# Autodesk Inventor assembly: Assembly1
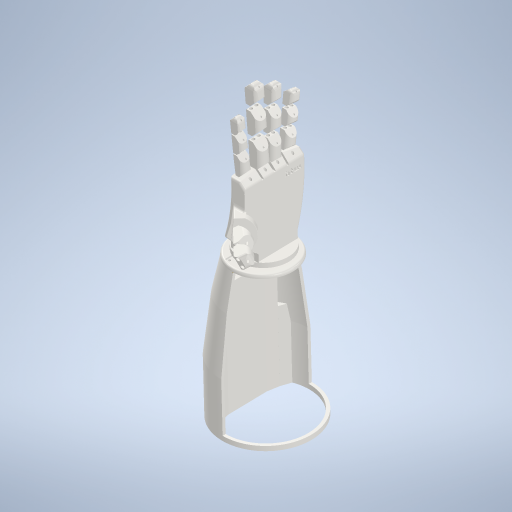
[picture p0: Inventor's stored thumbnail of the model, 512x512]
Saved by Autodesk Inventor 2024 (Build 280153000, 153)
## iProperties
Created: 2025-06-11
Part Number: Assembly1
Document SubType Name: Assembly
Designer: Mehdi Charfeddine
Author: Mehdi Charfeddine
## Documents named in this file (8)
- C:\Users\Mehdi Charfeddine\OneDrive\Bureau\original 3d\Assembly1.iam
- C:\Users\Mehdi Charfeddine\OneDrive\Bureau\original 3d\hand update.ipt
- C:\Users\Mehdi Charfeddine\OneDrive\Bureau\original 3d\update arm.ipt
- C:\Users\Mehdi Charfeddine\OneDrive\Bureau\original 3d\Daumen.ipt
- C:\Users\Mehdi Charfeddine\OneDrive\Bureau\original 3d\Zeigefinger.ipt
- C:\Users\Mehdi Charfeddine\OneDrive\Bureau\original 3d\Mittelfinger.ipt
- C:\Users\Mehdi Charfeddine\OneDrive\Bureau\original 3d\Ringfinger.ipt
- C:\Users\Mehdi Charfeddine\OneDrive\Bureau\original 3d\Kleiner Finger.ipt
## Components (7 placed, 7 different names)
1. hand update:1 — Mate:1, Mate:2, Mate:3, Mate:4, Mate:5, Mate:6
2. update arm:1 — Mate:1
3. Daumen:1 — Mate:2
4. Zeigefinger:1 — Mate:3
5. Mittelfinger:1 — Mate:4
6. Ringfinger:1 — Mate:5
7. Kleiner Finger:1 — Mate:6
## Relationships (6: Mate 6)
- Mate:1: hand update:1 ↔ update arm:1
- Mate:2: hand update:1 ↔ Daumen:1
- Mate:3: hand update:1 ↔ Zeigefinger:1
- Mate:4: hand update:1 ↔ Mittelfinger:1
- Mate:5: hand update:1 ↔ Ringfinger:1
- Mate:6: hand update:1 ↔ Kleiner Finger:1
